# Autodesk Inventor assembly: FE-130 End-Cap
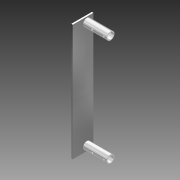
[picture p0: Inventor's stored thumbnail of the model, 180x180]
Saved by Autodesk Inventor 2021 (Build 250183000, 183)
## iProperties
Created: 2021-01-11
Part Number: FE-130 End-Cap
Document SubType Name: Assembly
## Documents named in this file (5)
- D:\FIRST\Design\FRC Fields\Generic Field Base\FE-100 Side Wall\FE-130 End-Cap\FE-130 End-Cap.iam
- D:\FIRST\Design\FRC Fields\Generic Field Base\FE-100 Side Wall\FE-130 End-Cap\FE-130-001 End Platet.ipt
- D:\FIRST\Design\FRC Fields\Generic Field Base\FE-100 Side Wall\FE-130 End-Cap\FE-130-003 Insert.ipt
- D:\FIRST\Design\FRC Fields\Generic Field Base\FE-100 Side Wall\FE-130 End-Cap\FE-130-002 End Tube.ipt
- D:\FIRST\Design\FRC Fields\Generic Field Base\FE-100 Side Wall\FE-130 End-Cap\FE-130-004 End Tube Mount.ipt
## Components (5 placed, 4 different names)
1. FE-130-001 End Platet:1 — Mate:1, Mate:2, Mate:4, Flush:3, Mate:6, Flush:5
2. FE-130-003 Insert:1 — Flush:1, Flush:2, Mate:1, Mate:2, Mate:3
3. FE-130-003 Insert:2 — Flush:1, Flush:2, Mate:3, Mate:4
4. FE-130-002 End Tube:1 — Flush:3, Tangent:1, Mate:5, Flush:4
5. FE-130-004 End Tube Mount:1 — Tangent:1, Mate:5, Flush:4, Mate:6, Flush:5
## Relationships (12: Mate 6, Flush 5, Tangent 1)
- Flush:1: FE-130-003 Insert:1 ↔ FE-130-003 Insert:2
- Flush:2: FE-130-003 Insert:1 ↔ FE-130-003 Insert:2
- Mate:1: FE-130-001 End Platet:1 ↔ FE-130-003 Insert:1
- Mate:2 (-21.4376 mm): FE-130-001 End Platet:1 ↔ FE-130-003 Insert:1
- Mate:3 (459.1749 mm): FE-130-003 Insert:1 ↔ FE-130-003 Insert:2
- Mate:4 (-27.7876 mm): FE-130-001 End Platet:1 ↔ FE-130-003 Insert:2
- Flush:3 (63.5 mm): FE-130-001 End Platet:1 ↔ FE-130-002 End Tube:1
- Tangent:1: FE-130-002 End Tube:1 ↔ FE-130-004 End Tube Mount:1
- Mate:5: FE-130-002 End Tube:1 ↔ FE-130-004 End Tube Mount:1
- Flush:4: FE-130-002 End Tube:1 ↔ FE-130-004 End Tube Mount:1
- Mate:6: FE-130-001 End Platet:1 ↔ FE-130-004 End Tube Mount:1
- Flush:5 (15.4432 mm): FE-130-001 End Platet:1 ↔ FE-130-004 End Tube Mount:1
